# Autodesk Inventor assembly: SidePanelFans
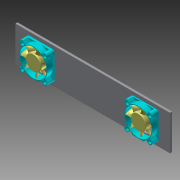
[picture p0: Inventor's stored thumbnail of the model, 180x180]
Saved by Autodesk Inventor 2015 (Build 190159000, 159)
## iProperties
Created: 2014-08-06
Part Number: SidePanelFans
Document SubType Name: Assembly
Designer: Patrick Camilleri
Author: Patrick Camilleri
## Documents named in this file (3)
- C:\Users\Patrick Camilleri\CAD\Test Box\SidePanelFans.iam
- C:\Users\Patrick Camilleri\CAD\Test Box\panel.ipt
- C:\Users\Patrick Camilleri\CAD\Models\CPU - -KF0410-01 - 40MM X 40MM X 10MM\Imported Components\CPU - -KF0410-01\CPU - -KF0410-01.iam
## Components (3 placed, 2 different names)
1. panel:1 — Cylindrical:1, Rigid:1
2. CPU - -KF0410-01:1 [sub-assembly] — Cylindrical:1
3. CPU - -KF0410-01:2 [sub-assembly] — Rigid:1
## Relationships (2: CylindricalJoint 1, WeldJoint 1)
- Cylindrical:1: panel:1 ↔ CPU - -KF0410-01:1
- Rigid:1 [WeldJoint]: panel:1 ↔ CPU - -KF0410-01:2
